# Autodesk Inventor assembly: Front_Panel_Base_Assembly
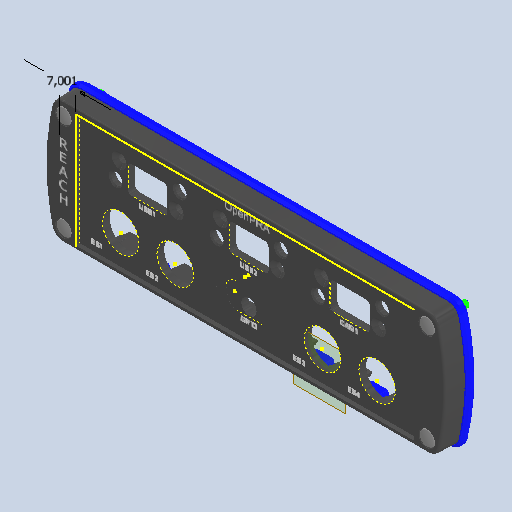
[picture p0: Inventor's stored thumbnail of the model, 512x512]
Saved by Autodesk Inventor 2022 (Build 260153000, 153)
## iProperties
Created: 2020-07-14
Part Number: Front_Panel_Base_Assembly
Document SubType Name: Assembly
Designer: CASE-SMALL2
Author: CASE-SMALL2
## Documents named in this file (7)
- C:\Users\Viktor\Google Drive\Unicorn 2020\CAD_V2\Front_Panel\Panel\Front_Panel_Base_Assembly.iam
- C:\Users\Viktor\Google Drive\Unicorn 2020\CAD_V2\Back_Panel\Panel\DI 1600.ipt
- C:\Users\Viktor\Google Drive\Unicorn 2020\CAD_V2\Back_Panel\Panel\SHR Z KT30X10 WN 1452 OG_3DSYM.ipt
- C:\Users\Viktor\Google Drive\Unicorn 2020\CAD_V2\Back_Panel\Panel\1009410_3D.ipt
- C:\Users\Viktor\Google Drive\Unicorn 2020\CAD_V2\Front_Panel\Panel\1009799_3D_Front.ipt
- C:\Users\Viktor\Google Drive\Unicorn 2020\CAD_V2\Front_Panel\Panel\1009799_3D_Front_CAM_version.ipt
- C:\Users\Viktor\Google Drive\Unicorn 2020\CAD_V2\Front_Panel\Panel\1009799_3D_Front_WaveRunner.ipt
## Components (12 placed, 6 different names)
1. 1009799_3D_Front:1 — Rigid:1, Rigid:2, Rigid:3, Rigid:4, Rigid:5, Rigid:6, Rigid:7, Rigid:8, Rigid:9
2. 1009799_3D_Front_CAM_version:1 — Rigid:9
3. 1009799_3D_Front_WaveRunner:1
4. DI 1600:1
5. SHR Z KT30X10 WN 1452 OG_3DSYM:1 — Rigid:1
6. SHR Z KT30X10 WN 1452 OG_3DSYM:2 — Rigid:5
7. SHR Z KT30X10 WN 1452 OG_3DSYM:3 — Rigid:3
8. SHR Z KT30X10 WN 1452 OG_3DSYM:4 — Rigid:7
9. 1009410_3D:1 — Rigid:2
10. 1009410_3D:2 — Rigid:4
11. 1009410_3D:3 — Rigid:8
12. 1009410_3D:4 — Rigid:6
## Relationships (10: WeldJoint 10)
- Rigid:1 [WeldJoint]: 1009799_3D_Front:1 ↔ SHR Z KT30X10 WN 1452 OG_3DSYM:1
- Rigid:2 [WeldJoint]: 1009799_3D_Front:1 ↔ 1009410_3D:1
- Rigid:3 [WeldJoint]: 1009799_3D_Front:1 ↔ SHR Z KT30X10 WN 1452 OG_3DSYM:3
- Rigid:4 [WeldJoint]: 1009799_3D_Front:1 ↔ 1009410_3D:2
- Rigid:5 [WeldJoint]: 1009799_3D_Front:1 ↔ SHR Z KT30X10 WN 1452 OG_3DSYM:2
- Rigid:6 [WeldJoint]: 1009799_3D_Front:1 ↔ 1009410_3D:4
- Rigid:7 [WeldJoint]: 1009799_3D_Front:1 ↔ SHR Z KT30X10 WN 1452 OG_3DSYM:4
- Rigid:8 [WeldJoint]: 1009799_3D_Front:1 ↔ 1009410_3D:3
- Rigid:9 [WeldJoint]: 1009799_3D_Front:1 ↔ 1009799_3D_Front_CAM_version:1
- [WeldJoint]: 1009799_3D_Front_CAM_version:1 ↔ 1009799_3D_Front_WaveRunner:1
